# Autodesk Inventor assembly: Assembly_Cube_v4
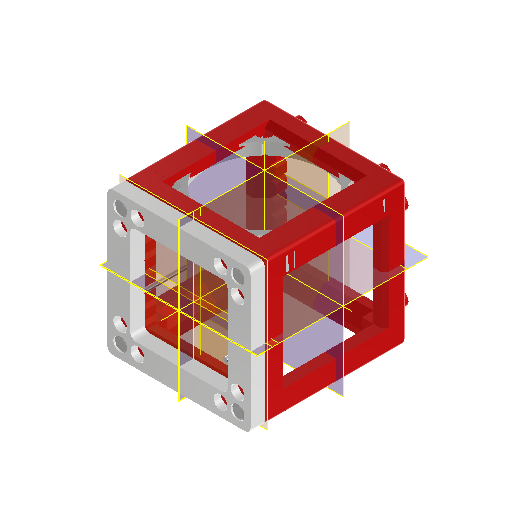
[picture p0: Inventor's stored thumbnail of the model, 512x512]
Saved by Autodesk Inventor 2025.1 (Build 291241020, 241B)
## iProperties
Created: 2024-08-17
Part Number: Assembly_Cube_v4
Document SubType Name: Assembly
Designer: diederichbenedict
Author: diederichbenedict
## Documents named in this file (7)
- C:\Users\diederichbenedict\Dropbox\Dokumente\Promotion\PROJECTS\TechnicalDocs-openUC2-QBox\Production_Files\CAD_Files\INVENTOR\Assembly_Cube_v4.iam
- C:\Users\diederichbenedict\Dropbox\Dokumente\Promotion\PROJECTS\TechnicalDocs-openUC2-QBox\Production_Files\CAD_Files\INVENTOR\10_Cube_v4.ipt
- C:\Users\diederichbenedict\Dropbox\Dokumente\Promotion\PROJECTS\TechnicalDocs-openUC2-QBox\Production_Files\CAD_Files\INVENTOR\10_Insert_v4.ipt
- C:\Users\diederichbenedict\Dropbox\Dokumente\Promotion\PROJECTS\TechnicalDocs-openUC2-QBox\Production_Files\CAD_Files\INVENTOR\00_ballmagnet_5mm.ipt
- C:\Users\diederichbenedict\Dropbox\Dokumente\Promotion\PROJECTS\TechnicalDocs-openUC2-QBox\Production_Files\CAD_Files\INVENTOR\00_pins_1.5mmx14mm.ipt
- C:\Users\diederichbenedict\Dropbox\Dokumente\Promotion\PROJECTS\TechnicalDocs-openUC2-QBox\Production_Files\CAD_Files\INVENTOR\10_Base_v4.ipt
- C:\Users\diederichbenedict\Dropbox\Dokumente\Promotion\PROJECTS\TechnicalDocs-openUC2-QBox\Production_Files\CAD_Files\INVENTOR\DIN 913 - M5 x 5.ipt
## Components (14 placed, 6 different names)
1. 10_Cube_v4:1 — Mate:1, Tangent:1, Flush:4, Flush:7, Flush:8, Mate:2, Mate:3
2. 10_Base_v4:1 — Flush:3, Flush:4, Insert:2, Insert:3, Insert:4, Insert:5
3. DIN 913 - M5 x 5:1 — Insert:4
4. DIN 913 - M5 x 5:2 — Insert:3
5. DIN 913 - M5 x 5:3 — Insert:2
6. DIN 913 - M5 x 5:4 — Insert:5
7. 00_pins_1.5mmx14mm:1
8. 10_Insert_v4:1 — Flush:7, Flush:8
9. 00_pins_1.5mmx14mm:2
10. 10_Cube_v4:2 — Mate:2, Mate:3
11. 00_ballmagnet_5mm:1 — Mate:1, Tangent:1
12. 00_ballmagnet_5mm:2
13. 00_ballmagnet_5mm:3
14. 00_ballmagnet_5mm:4
## Component patterns: (4 elements, first: 00_ballmagnet_5mm:1)
## Relationships (12: Flush 4, Insert 4, Mate 3, Tangent 1)
- Mate:1: 10_Cube_v4:1 ↔ 00_ballmagnet_5mm:1
- Tangent:1: 10_Cube_v4:1 ↔ 00_ballmagnet_5mm:1
- Flush:3: 10_Base_v4:1
- Flush:4: 10_Cube_v4:1 ↔ 10_Base_v4:1
- Insert:2: 10_Base_v4:1 ↔ DIN 913 - M5 x 5:3
- Insert:3: 10_Base_v4:1 ↔ DIN 913 - M5 x 5:2
- Insert:4: 10_Base_v4:1 ↔ DIN 913 - M5 x 5:1
- Insert:5: 10_Base_v4:1 ↔ DIN 913 - M5 x 5:4
- Flush:7: 10_Cube_v4:1 ↔ 10_Insert_v4:1
- Flush:8: 10_Cube_v4:1 ↔ 10_Insert_v4:1
- Mate:2: 10_Cube_v4:1 ↔ 10_Cube_v4:2
- Mate:3: 10_Cube_v4:1 ↔ 10_Cube_v4:2
